# Autodesk Inventor assembly: CAR_010_Versa+Motor
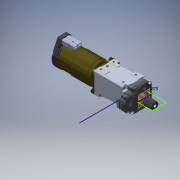
[picture p0: Inventor's stored thumbnail of the model, 180x180]
Saved by Autodesk Inventor 2018.3 (Build 223284000, 284)
## iProperties
Created: 2020-01-30
Part Number: CAR_010_Versa+Motor
Document SubType Name: Assembly
Designer: 22turnmaxw
Author: 22turnmaxw
## Documents named in this file (3)
- C:\Users\22barlalex\Documents\GrabCAD\Infinite Recharge 2020\Build season\CAR_010_Versa+Motor.iam
- C:\Users\22barlalex\Documents\GrabCAD\Infinite Recharge 2020\Brainstorming\Versaplanetary\775 Motor.ipt
- C:\Users\22barlalex\Documents\GrabCAD\Infinite Recharge 2020\Brainstorming\Versaplanetary\VersaPlanetary Gearbox.iam
## Components (2 placed, 2 different names)
1. 775 Motor:1 — Mate:1, Mate:2
2. VersaPlanetary Gearbox:1 [sub-assembly] — Mate:1, Mate:2
## Relationships (2: Mate 2)
- Mate:1: 775 Motor:1 ↔ VersaPlanetary Gearbox:1
- Mate:2: 775 Motor:1 ↔ VersaPlanetary Gearbox:1
